# Autodesk Inventor assembly: LEG2
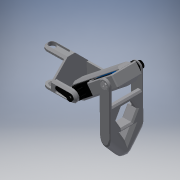
[picture p0: Inventor's stored thumbnail of the model, 180x180]
Saved by Autodesk Inventor 2017 (Build 210142000, 142)
## iProperties
Created: 2017-09-24
Part Number: LEG2
Document SubType Name: Assembly
Designer: Alexander Miller
Author: Alexander Miller
## Documents named in this file (7)
- X:\Alex\Documents\Git\HeRo-Mini\Hardware\LEG.iam
- X:\Alex\Documents\Git\HeRo-Mini\Hardware\SERVO.iam
- X:\Alex\Documents\Git\HeRo-Mini\Hardware\COXA.ipt
- X:\Alex\Documents\Git\HeRo-Mini\Hardware\FEMUR_A.ipt
- X:\Alex\Documents\Git\HeRo-Mini\Hardware\FEMUR_B.ipt
- X:\Alex\Documents\Git\HeRo-Mini\Hardware\BEARING.ipt
- X:\Alex\Documents\Git\HeRo-Mini\Hardware\TIBIA.ipt
## Components (10 placed, 6 different names)
1. SERVO:1 [sub-assembly] — Rigid:1, Rigid:3, Rigid:7
2. SERVO:2 [sub-assembly] — Rigid:2, Rigid:4, Rigid:6
3. COXA:1 — Rotational:1, Rotational:2, Rigid:7
4. FEMUR_A:1 — Rigid:1, Rigid:2
5. FEMUR_B:1 — Rigid:4
6. FEMUR_B:2 — Rigid:3
7. BEARING:1 — Rotational:1
8. BEARING:2 — Rotational:2
9. TIBIA:1 — Rotational:3, Rigid:6
10. BEARING:3 — Rotational:3
## Relationships (9: WeldJoint 6, RevoluteJoint 3)
- Rigid:1 [WeldJoint]: SERVO:1 ↔ FEMUR_A:1
- Rigid:2 [WeldJoint]: SERVO:2 ↔ FEMUR_A:1
- Rigid:3 [WeldJoint]: SERVO:1 ↔ FEMUR_B:2
- Rigid:4 [WeldJoint]: SERVO:2 ↔ FEMUR_B:1
- Rotational:1 [RevoluteJoint]: COXA:1 ↔ BEARING:1
- Rotational:2 [RevoluteJoint]: COXA:1 ↔ BEARING:2
- Rotational:3 [RevoluteJoint]: TIBIA:1 ↔ BEARING:3
- Rigid:6 [WeldJoint]: SERVO:2 ↔ TIBIA:1
- Rigid:7 [WeldJoint]: SERVO:1 ↔ COXA:1
